# Autodesk Inventor assembly: Neo_Led_Complette
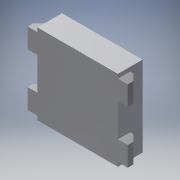
[picture p0: Inventor's stored thumbnail of the model, 180x180]
Saved by Autodesk Inventor 2017 (Build 210142000, 142)
## iProperties
Created: 2018-11-04
Part Number: Neo_Led_Complette
Document SubType Name: Assembly
Designer: ludov
Author: ludov
## Documents named in this file (3)
- C:\Users\ludov\Dropbox\Electronique\Vario\Hardware\V3.00\Neo_Led_Complette.iam
- C:\Users\ludov\Dropbox\Electronique\Vario\Hardware\V3.00\Nes_Led.ipt
- C:\Users\ludov\Dropbox\Electronique\Vario\Hardware\V3.00\Vitre led.ipt
## Components (2 placed, 2 different names)
1. Nes_Led:1 — Rotation:1
2. Vitre led:1 — Rotation:1
## Relationships (1: RevoluteJoint 1)
- Rotation:1 [RevoluteJoint]: Nes_Led:1 ↔ Vitre led:1
